# Autodesk Inventor assembly: Assembly1
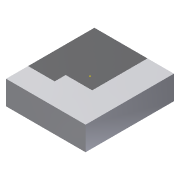
[picture p0: Inventor's stored thumbnail of the model, 180x180]
Saved by Autodesk Inventor 2015 (Build 190159000, 159)
## iProperties
Created: 2021-06-10
Part Number: Assembly1
Document SubType Name: Assembly
Designer: Mia
Author: Mia
## Documents named in this file (3)
- C:\Users\Mia\Desktop\MS\thesis\my thesis report\cube\Assembly1.iam
- C:\Users\Mia\Desktop\MS\thesis\my thesis report\cube\data.ipt
- C:\Users\Mia\Desktop\MS\thesis\my thesis report\cube\no_data.ipt
## Components (2 placed, 2 different names)
1. data:1 — Mate:1, Mate:2, Mate:3, Flush:1
2. no_data:1 — Mate:1, Mate:2, Mate:3, Flush:1
## Relationships (4: Mate 3, Flush 1)
- Mate:1: data:1 ↔ no_data:1
- Mate:2: data:1 ↔ no_data:1
- Mate:3: data:1 ↔ no_data:1
- Flush:1: data:1 ↔ no_data:1
